# Autodesk Inventor assembly: leg_tibea_ass
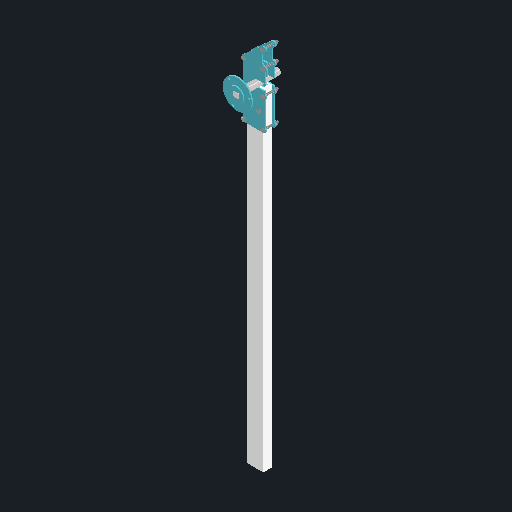
[picture p0: Inventor's stored thumbnail of the model, 512x512]
Saved by Autodesk Inventor 2026 (Build 300175000, 175)
## iProperties
Created: 2026-04-23
Part Number: leg_tibea_ass
Document SubType Name: Assembly
Designer: user
Mass: 1838.87 g
Surface Area: 2426.07 cm^2
Volume: 452.277 cm^3
Author: user
## Documents named in this file (16)
- C:\Users\user\vs_code_projects\ogonek-spider\physical-structure\cad\leg_tibea\leg_Right_tibea_ass.iam
- leg_Right_tibea_ass.iam
- C:\Users\user\vs_code_projects\ogonek-spider\physical-structure\cad\leg_tibea\tibea_profile.ipt
- C:\Users\user\vs_code_projects\ogonek-spider\physical-structure\cad\leg_tibea\tibea_inside_steel.ipt
- C:\Users\user\vs_code_projects\ogonek-spider\physical-structure\cad\leg_tibea\tibea_outside_steel.ipt
- C:\Users\user\vs_code_projects\ogonek-spider\physical-structure\cad\leg_tibea\shaft_tibea.ipt
- C:\Users\user\vs_code_projects\ogonek-spider\physical-structure\cad\leg_tibea\tibea_vodilo_steel.ipt
- C:\Users\user\Documents\Inventor\Content Center Files\R2026\ru-RU\GOST 7805-70\Болт M5-6gx35 ГОСТ 7805-70.ipt
- C:\Users\user\Documents\Inventor\Content Center Files\R2026\ru-RU\Nut GOST R 50592-93\Гайка M5-6H ГОСТ Р 50592-93.ipt
- C:\Users\user\vs_code_projects\ogonek-spider\physical-structure\cad\parametres.xlsx
- C:\Users\user\vs_code_projects\ogonek-spider\physical-structure\cad\leg_tibea\leg_Left_tibea_ass\AIP\FEA\fer4zszvk.fins
- C:\Users\user\vs_code_projects\ogonek-spider\physical-structure\cad\leg_tibea\leg_Left_tibea_ass\AIP\FEA\fer4zszvk.fsat
- C:\Users\user\vs_code_projects\ogonek-spider\physical-structure\cad\leg_tibea\leg_Left_tibea_ass\AIP\FEA\fer4zszvk.ftes
- C:\Users\user\vs_code_projects\ogonek-spider\physical-structure\cad\leg_tibea\leg_Left_tibea_ass\AIP\FEA\fer4zszvk.fwiz
- C:\Users\user\vs_code_projects\ogonek-spider\physical-structure\cad\leg_tibea\leg_Left_tibea_ass\AIP\FEA\fer4zszy8.fmsh
- C:\Users\user\vs_code_projects\ogonek-spider\physical-structure\cad\leg_tibea\leg_Left_tibea_ass\AIP\FEA\fer8dcvr4.fres
## Components (25 placed, 7 different names)
1. tibea_profile:1 — Жесткий:1, Жесткий:2, Жесткий:3, Жесткий:4
2. tibea_inside_steel:1 — Жесткий:1
3. tibea_inside_steel:2 — Жесткий:2
4. tibea_outside_steel:1 — Жесткий:3, Совмещение:1, Совмещение:2, Совмещение:3, Совмещение:4, Совмещение:5, Совмещение:6, Совмещение:7, Совмещение:8, Совмещение:9, Совмещение:10, Совмещение:11, Совмещение:12, Совмещение:13, Совмещение:14, Совмещение:15, Совмещение:16, Совмещение:17, Совмещение:18, Совмещение:19, Совмещение:21, Совмещение:23, Совмещение:25, Совмещение:27, Совмещение:29, Совмещение:31, Совмещение:33, Совмещение:35, Жесткий:11
5. tibea_outside_steel:2 — Жесткий:4, Совмещение:20, Совмещение:22, Совмещение:24, Совмещение:26, Совмещение:28, Совмещение:30, Совмещение:32, Совмещение:34, Совмещение:36
6. shaft_tibea:1 — Жесткий:10, Жесткий:11
7. tibea_vodilo_steel:1 — Жесткий:10
8. Болт ГОСТ 7805-70 M5-6gx35:1 — Совмещение:1, Совмещение:2
9. Гайка ГОСТ Р 50592-93 M5:1 — Совмещение:19, Совмещение:20
10. Болт ГОСТ 7805-70 M5-6gx35:2 — Совмещение:3, Совмещение:4
11. Болт ГОСТ 7805-70 M5-6gx35:3 — Совмещение:5, Совмещение:6
12. Болт ГОСТ 7805-70 M5-6gx35:4 — Совмещение:7, Совмещение:8
13. Болт ГОСТ 7805-70 M5-6gx35:5 — Совмещение:9, Совмещение:10
14. Болт ГОСТ 7805-70 M5-6gx35:6 — Совмещение:11, Совмещение:12
15. Болт ГОСТ 7805-70 M5-6gx35:7 — Совмещение:13, Совмещение:14
16. Болт ГОСТ 7805-70 M5-6gx35:8 — Совмещение:15, Совмещение:16
17. Болт ГОСТ 7805-70 M5-6gx35:9 — Совмещение:17, Совмещение:18
18. Гайка ГОСТ Р 50592-93 M5:2 — Совмещение:21, Совмещение:22
19. Гайка ГОСТ Р 50592-93 M5:3 — Совмещение:23, Совмещение:24
20. Гайка ГОСТ Р 50592-93 M5:4 — Совмещение:25, Совмещение:26
21. Гайка ГОСТ Р 50592-93 M5:5 — Совмещение:27, Совмещение:28
22. Гайка ГОСТ Р 50592-93 M5:6 — Совмещение:29, Совмещение:30
23. Гайка ГОСТ Р 50592-93 M5:7 — Совмещение:31, Совмещение:32
24. Гайка ГОСТ Р 50592-93 M5:8 — Совмещение:33, Совмещение:34
25. Гайка ГОСТ Р 50592-93 M5:9 — Совмещение:35, Совмещение:36
## Relationships (42: Mate 36, WeldJoint 6)
- Жесткий:1 [WeldJoint]: tibea_profile:1 ↔ tibea_inside_steel:1
- Жесткий:2 [WeldJoint]: tibea_profile:1 ↔ tibea_inside_steel:2
- Жесткий:3 [WeldJoint]: tibea_profile:1 ↔ tibea_outside_steel:1
- Жесткий:4 [WeldJoint]: tibea_profile:1 ↔ tibea_outside_steel:2
- Жесткий:10 [WeldJoint]: shaft_tibea:1 ↔ tibea_vodilo_steel:1
- Совмещение:1 [Mate]: tibea_outside_steel:1 ↔ Болт ГОСТ 7805-70 M5-6gx35:1
- Совмещение:2 [Mate]: tibea_outside_steel:1 ↔ Болт ГОСТ 7805-70 M5-6gx35:1
- Совмещение:3 [Mate]: tibea_outside_steel:1 ↔ Болт ГОСТ 7805-70 M5-6gx35:2
- Совмещение:4 [Mate]: tibea_outside_steel:1 ↔ Болт ГОСТ 7805-70 M5-6gx35:2
- Совмещение:5 [Mate]: tibea_outside_steel:1 ↔ Болт ГОСТ 7805-70 M5-6gx35:3
- Совмещение:6 [Mate]: tibea_outside_steel:1 ↔ Болт ГОСТ 7805-70 M5-6gx35:3
- Совмещение:7 [Mate]: tibea_outside_steel:1 ↔ Болт ГОСТ 7805-70 M5-6gx35:4
- Совмещение:8 [Mate]: tibea_outside_steel:1 ↔ Болт ГОСТ 7805-70 M5-6gx35:4
- Совмещение:9 [Mate]: tibea_outside_steel:1 ↔ Болт ГОСТ 7805-70 M5-6gx35:5
- Совмещение:10 [Mate]: tibea_outside_steel:1 ↔ Болт ГОСТ 7805-70 M5-6gx35:5
- Совмещение:11 [Mate]: tibea_outside_steel:1 ↔ Болт ГОСТ 7805-70 M5-6gx35:6
- Совмещение:12 [Mate]: tibea_outside_steel:1 ↔ Болт ГОСТ 7805-70 M5-6gx35:6
- Совмещение:13 [Mate]: tibea_outside_steel:1 ↔ Болт ГОСТ 7805-70 M5-6gx35:7
- Совмещение:14 [Mate]: tibea_outside_steel:1 ↔ Болт ГОСТ 7805-70 M5-6gx35:7
- Совмещение:15 [Mate]: tibea_outside_steel:1 ↔ Болт ГОСТ 7805-70 M5-6gx35:8
- Совмещение:16 [Mate]: tibea_outside_steel:1 ↔ Болт ГОСТ 7805-70 M5-6gx35:8
- Совмещение:17 [Mate]: tibea_outside_steel:1 ↔ Болт ГОСТ 7805-70 M5-6gx35:9
- Совмещение:18 [Mate]: tibea_outside_steel:1 ↔ Болт ГОСТ 7805-70 M5-6gx35:9
- Совмещение:19 [Mate]: tibea_outside_steel:1 ↔ Гайка ГОСТ Р 50592-93 M5:1
- Совмещение:20 [Mate]: tibea_outside_steel:2 ↔ Гайка ГОСТ Р 50592-93 M5:1
- Совмещение:21 [Mate]: tibea_outside_steel:1 ↔ Гайка ГОСТ Р 50592-93 M5:2
- Совмещение:22 [Mate]: tibea_outside_steel:2 ↔ Гайка ГОСТ Р 50592-93 M5:2
- Совмещение:23 [Mate]: tibea_outside_steel:1 ↔ Гайка ГОСТ Р 50592-93 M5:3
- Совмещение:24 [Mate]: tibea_outside_steel:2 ↔ Гайка ГОСТ Р 50592-93 M5:3
- Совмещение:25 [Mate]: tibea_outside_steel:1 ↔ Гайка ГОСТ Р 50592-93 M5:4
- Совмещение:26 [Mate]: tibea_outside_steel:2 ↔ Гайка ГОСТ Р 50592-93 M5:4
- Совмещение:27 [Mate]: tibea_outside_steel:1 ↔ Гайка ГОСТ Р 50592-93 M5:5
- Совмещение:28 [Mate]: tibea_outside_steel:2 ↔ Гайка ГОСТ Р 50592-93 M5:5
- Совмещение:29 [Mate]: tibea_outside_steel:1 ↔ Гайка ГОСТ Р 50592-93 M5:6
- Совмещение:30 [Mate]: tibea_outside_steel:2 ↔ Гайка ГОСТ Р 50592-93 M5:6
- Совмещение:31 [Mate]: tibea_outside_steel:1 ↔ Гайка ГОСТ Р 50592-93 M5:7
- Совмещение:32 [Mate]: tibea_outside_steel:2 ↔ Гайка ГОСТ Р 50592-93 M5:7
- Совмещение:33 [Mate]: tibea_outside_steel:1 ↔ Гайка ГОСТ Р 50592-93 M5:8
- Совмещение:34 [Mate]: tibea_outside_steel:2 ↔ Гайка ГОСТ Р 50592-93 M5:8
- Совмещение:35 [Mate]: tibea_outside_steel:1 ↔ Гайка ГОСТ Р 50592-93 M5:9
- Совмещение:36 [Mate]: tibea_outside_steel:2 ↔ Гайка ГОСТ Р 50592-93 M5:9
- Жесткий:11 [WeldJoint]: tibea_outside_steel:1 ↔ shaft_tibea:1
## Named parameters: tolerance_plazma = 0.1 mm, thickness_steel = 3 mm, d_main_screw_holes = 6.1 mm, d_main_shaft = 16 mm, thickness_profile_tibea = 4 mm, width_profile_tibea = 20 mm, hight_profile_tibea = 40 mm, length_profile_tibia = 800 mm, length_thorn_tibia = 400 mm, width_shaft_shift = 35 mm, length_profile_femur = 350 mm, thickness_profile_femur = 3 mm, width_profile_femur = 50 mm, hight_shaft_shift = 40 mm, hight_profile_femur = 50 mm, width_flattened_surface = 12 mm, sa_0 = 1.6e+06, length_coxa = 100 mm, hight_coxa = 40 mm, width_coxa = 80 mm, width_body_l1 = 100 mm, width_body_l2 = 150 mm, width_body_l3 = 120 mm, offset_body_l12 = 60 mm, offset_body_l12_1 = 200 mm, offset_body_l23 = 200 mm, hight_ground_clearance = 500 mm
note: some values were not read from the file. Shown as the stored number, unit unknown: "sa_0".
